# Autodesk Inventor assembly: Sheathing_For_Side
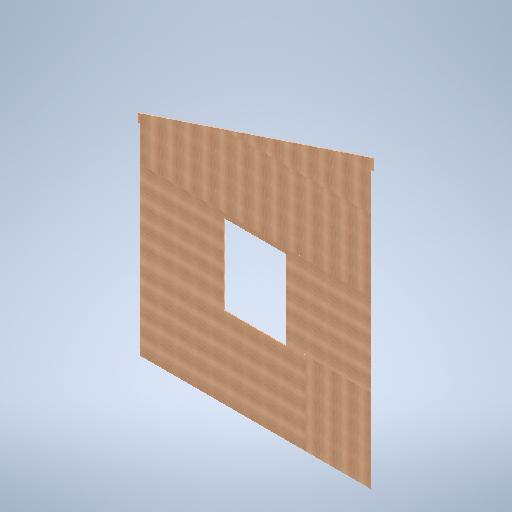
[picture p0: Inventor's stored thumbnail of the model, 512x512]
Saved by Autodesk Inventor 2025.1 (Build 291241020, 241B)
## iProperties
Created: 2024-10-03
Part Number: Sheathing_For_Side
Document SubType Name: Assembly
Designer: Tom
Author: Tom
## Documents named in this file (8)
- C:\Users\Tom\Documents\Inventor\Mobility\Additional_Building\Sheathing_For_Side.iam
- C:\Users\Tom\Documents\Inventor\Mobility\Additional_Building\OSB_For_Walls_With_Dimensions_48_x_96_Inches.ipt
- C:\Users\Tom\Documents\Inventor\Mobility\Additional_Building\OSB_For_Walls_With_Dimensions_48_x_48_Inches.ipt
- C:\Users\Tom\Documents\Inventor\Mobility\Additional_Building\OSB_For_Walls_With_Dimensions_48_x_85_Inches.ipt
- C:\Users\Tom\Documents\Inventor\Mobility\Additional_Building\OSB_For_Walls_With_Dimensions_38.375_x_40.979_Inches.ipt
- C:\Users\Tom\Documents\Inventor\Mobility\Additional_Building\OSB_For_Walls_With_Dimensions_37_x_48_Inches.ipt
- C:\Users\Tom\Documents\Inventor\Mobility\Additional_Building\OSB_For_Side_And_Back.ipt
- C:\Users\Tom\Documents\Inventor\Mobility\Additional_Building\OSB_For_Side_And_Top.ipt
## Components (7 placed, 7 different names)
1. OSB_For_Walls_With_Dimensions_48_x_96_Inches:1 — Mate:1, Mate:2, Mate:3, Mate:5, Flush:3, Flush:4, Flush:11, Flush:12, Mate:12, Mate:13, Flush:20, Flush:21, Flush:22
2. OSB_For_Walls_With_Dimensions_48_x_48_Inches:1 — Mate:5, Flush:3, Flush:4, Mate:7, Flush:11, Flush:15, Flush:22, Mate:18
3. OSB_For_Walls_With_Dimensions_48_x_85_Inches:1 — Mate:7, Flush:12, Flush:15, Mate:11, Mate:13, Flush:21, Mate:17, Flush:26, Flush:27
4. OSB_For_Walls_With_Dimensions_37_x_48_Inches:1 — Mate:11, Mate:12, Flush:20
5. OSB_For_Walls_With_Dimensions_38.375_x_40.979_Inches:1 — Mate:17, Flush:26, Flush:27, Mate:19, Flush:28, Flush:30
6. OSB_For_Side_And_Back:1 — Mate:18, Mate:19, Flush:28, Mate:20, Flush:29
7. OSB_For_Side_And_Top:1 — Mate:20, Flush:29, Flush:30
## Relationships (25: Flush 13, Mate 12)
- Mate:1: OSB_For_Walls_With_Dimensions_48_x_96_Inches:1
- Mate:2: OSB_For_Walls_With_Dimensions_48_x_96_Inches:1
- Mate:3: OSB_For_Walls_With_Dimensions_48_x_96_Inches:1
- Mate:5: OSB_For_Walls_With_Dimensions_48_x_96_Inches:1 ↔ OSB_For_Walls_With_Dimensions_48_x_48_Inches:1
- Flush:3: OSB_For_Walls_With_Dimensions_48_x_96_Inches:1 ↔ OSB_For_Walls_With_Dimensions_48_x_48_Inches:1
- Flush:4: OSB_For_Walls_With_Dimensions_48_x_96_Inches:1 ↔ OSB_For_Walls_With_Dimensions_48_x_48_Inches:1
- Mate:7: OSB_For_Walls_With_Dimensions_48_x_48_Inches:1 ↔ OSB_For_Walls_With_Dimensions_48_x_85_Inches:1
- Flush:11: OSB_For_Walls_With_Dimensions_48_x_96_Inches:1 ↔ OSB_For_Walls_With_Dimensions_48_x_48_Inches:1
- Flush:12: OSB_For_Walls_With_Dimensions_48_x_96_Inches:1 ↔ OSB_For_Walls_With_Dimensions_48_x_85_Inches:1
- Flush:15: OSB_For_Walls_With_Dimensions_48_x_48_Inches:1 ↔ OSB_For_Walls_With_Dimensions_48_x_85_Inches:1
- Mate:11: OSB_For_Walls_With_Dimensions_48_x_85_Inches:1 ↔ OSB_For_Walls_With_Dimensions_37_x_48_Inches:1
- Mate:12: OSB_For_Walls_With_Dimensions_48_x_96_Inches:1 ↔ OSB_For_Walls_With_Dimensions_37_x_48_Inches:1
- Mate:13: OSB_For_Walls_With_Dimensions_48_x_96_Inches:1 ↔ OSB_For_Walls_With_Dimensions_48_x_85_Inches:1
- Flush:20: OSB_For_Walls_With_Dimensions_48_x_96_Inches:1 ↔ OSB_For_Walls_With_Dimensions_37_x_48_Inches:1
- Flush:21: OSB_For_Walls_With_Dimensions_48_x_96_Inches:1 ↔ OSB_For_Walls_With_Dimensions_48_x_85_Inches:1
- Flush:22: OSB_For_Walls_With_Dimensions_48_x_96_Inches:1 ↔ OSB_For_Walls_With_Dimensions_48_x_48_Inches:1
- Mate:17: OSB_For_Walls_With_Dimensions_48_x_85_Inches:1 ↔ OSB_For_Walls_With_Dimensions_38.375_x_40.979_Inches:1
- Flush:26: OSB_For_Walls_With_Dimensions_48_x_85_Inches:1 ↔ OSB_For_Walls_With_Dimensions_38.375_x_40.979_Inches:1
- Flush:27: OSB_For_Walls_With_Dimensions_48_x_85_Inches:1 ↔ OSB_For_Walls_With_Dimensions_38.375_x_40.979_Inches:1
- Mate:18: OSB_For_Walls_With_Dimensions_48_x_48_Inches:1 ↔ OSB_For_Side_And_Back:1
- Mate:19: OSB_For_Walls_With_Dimensions_38.375_x_40.979_Inches:1 ↔ OSB_For_Side_And_Back:1
- Flush:28: OSB_For_Walls_With_Dimensions_38.375_x_40.979_Inches:1 ↔ OSB_For_Side_And_Back:1
- Mate:20: OSB_For_Side_And_Back:1 ↔ OSB_For_Side_And_Top:1
- Flush:29: OSB_For_Side_And_Back:1 ↔ OSB_For_Side_And_Top:1
- Flush:30: OSB_For_Walls_With_Dimensions_38.375_x_40.979_Inches:1 ↔ OSB_For_Side_And_Top:1
